# Autodesk Inventor assembly: Поворотный узел схвата
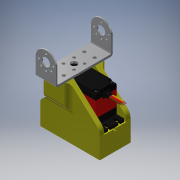
[picture p0: Inventor's stored thumbnail of the model, 180x180]
Saved by Autodesk Inventor 2019.1 (Build 231200000, 200)
## iProperties
Created: 2018-10-15
Part Number: Поворотный узел схвата
Material: Типовые
Document SubType Name: Assembly
Designer: Олег
Author: Олег
## Documents named in this file (5)
- C:\Users\Олег\OneDrive\Общая\NoSpace 2.0\Манипулятор\Поворотный узел схвата\Поворотный узел схвата.iam
- C:\Users\Олег\OneDrive\Общая\NoSpace 2.0\Манипулятор\PDI 6621MG.ipt
- C:\Users\Олег\OneDrive\Общая\NoSpace 2.0\Манипулятор\Поворотный узел схвата\Подшипниковый блок поворотного узла схвата.ipt
- C:\Users\Олег\OneDrive\Общая\NoSpace 2.0\Манипулятор\Поворотный узел схвата\Подшипник 17х26х5.ipt
- C:\Users\Олег\OneDrive\Общая\NoSpace 2.0\Манипулятор\Servoarm 2 RDS3115.ipt
## Components (4 placed, 4 different names)
1. PDI 6621MG:1 — Совмещение:2, Совмещение:3, Совмещение:4
2. Подшипниковый блок поворотного узла схвата:1 — Совмещение:1, Заподлицо:1, Совмещение:2, Совмещение:3, Совмещение:4, Совмещение:5, Совмещение:6, Совмещение:7
3. Подшипник 17х26х5:1 — Совмещение:1, Заподлицо:1
4. Servoarm 2 RDS3115:1 — Совмещение:5, Совмещение:6, Совмещение:7
## Relationships (8: Mate 7, Flush 1)
- Совмещение:1 [Mate]: Подшипниковый блок поворотного узла схвата:1 ↔ Подшипник 17х26х5:1
- Заподлицо:1 [Flush]: Подшипниковый блок поворотного узла схвата:1 ↔ Подшипник 17х26х5:1
- Совмещение:2 [Mate]: PDI 6621MG:1 ↔ Подшипниковый блок поворотного узла схвата:1
- Совмещение:3 [Mate]: PDI 6621MG:1 ↔ Подшипниковый блок поворотного узла схвата:1
- Совмещение:4 [Mate]: PDI 6621MG:1 ↔ Подшипниковый блок поворотного узла схвата:1
- Совмещение:5 [Mate]: Подшипниковый блок поворотного узла схвата:1 ↔ Servoarm 2 RDS3115:1
- Совмещение:6 [Mate]: Подшипниковый блок поворотного узла схвата:1 ↔ Servoarm 2 RDS3115:1
- Совмещение:7 [Mate]: Подшипниковый блок поворотного узла схвата:1 ↔ Servoarm 2 RDS3115:1
